# Autodesk Inventor assembly: Zusammengesetzt_2_Rechen_neu_3D
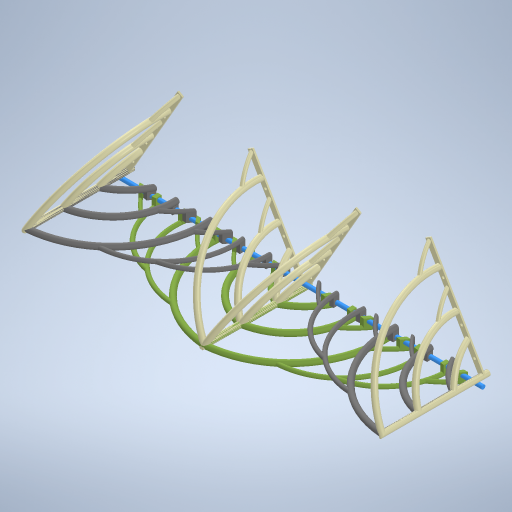
[picture p0: Inventor's stored thumbnail of the model, 512x512]
Saved by Autodesk Inventor 2024 (Build 280153000, 153)
## iProperties
Created: 2023-12-09
Part Number: Zusammengesetzt_2_Rechen_neu_3D
Document SubType Name: Assembly
Designer: mikao
Author: mikao
## Documents named in this file (5)
- \\192.168.122.200\studenten_bionik\Austausch\MikaOhler\Inventormodelle\Zusammengesetzt_2_Rechen_Stern_3D_Dickere_Wurzeln.iam
- \\192.168.122.200\studenten_bionik\Austausch\MikaOhler\Inventormodelle\schubsicherung_modul_links_Boden_glatt.ipt
- \\192.168.122.200\studenten_bionik\Austausch\MikaOhler\Inventormodelle\schubsicherung_modul_links_Boden_glatt_MIR.ipt
- \\192.168.122.200\studenten_bionik\Austausch\MikaOhler\Inventormodelle\schubsicherung_modul_links_Boden_glatt_Stütze.ipt
- \\192.168.122.200\studenten_bionik\Austausch\MikaOhler\Inventormodelle\Stange_4_Rechen.ipt
## Components (11 placed, 4 different names)
1. schubsicherung_modul_links_Boden_glatt:1 — Fluchtend:1, Starr:1
2. schubsicherung_modul_links_Boden_glatt:2 — Drehbar:1
3. schubsicherung_modul_links_Boden_glatt_MIR:1 — Passend:1, Drehbar:5
4. schubsicherung_modul_links_Boden_glatt_MIR:2 — Drehbar:3
5. schubsicherung_modul_links_Boden_glatt_Stütze:1 — Drehbar:1, Drehbar:2
6. schubsicherung_modul_links_Boden_glatt_Stütze:2 — Drehbar:4
7. Stange_4_Rechen:1 — Starr:1
8. schubsicherung_modul_links_Boden_glatt_Stütze:3 — Drehbar:2
9. schubsicherung_modul_links_Boden_glatt_Stütze:4 — Drehbar:3, Drehbar:4
10. schubsicherung_modul_links_Boden_glatt_Stütze:5 — Drehbar:5, Drehbar:6
11. schubsicherung_modul_links_Boden_glatt_Stütze:6 — Drehbar:6
## Relationships (9: RevoluteJoint 6, Flush 1, Mate 1, WeldJoint 1)
- Fluchtend:1 [Flush]: schubsicherung_modul_links_Boden_glatt:1
- Passend:1 [Mate]: schubsicherung_modul_links_Boden_glatt_MIR:1
- Starr:1 [WeldJoint] (54.55 mm): schubsicherung_modul_links_Boden_glatt:1 ↔ Stange_4_Rechen:1
- Drehbar:1 [RevoluteJoint]: schubsicherung_modul_links_Boden_glatt:2 ↔ schubsicherung_modul_links_Boden_glatt_Stütze:1
- Drehbar:2 [RevoluteJoint]: schubsicherung_modul_links_Boden_glatt_Stütze:1 ↔ schubsicherung_modul_links_Boden_glatt_Stütze:3
- Drehbar:3 [RevoluteJoint]: schubsicherung_modul_links_Boden_glatt_MIR:2 ↔ schubsicherung_modul_links_Boden_glatt_Stütze:4
- Drehbar:4 [RevoluteJoint]: schubsicherung_modul_links_Boden_glatt_Stütze:2 ↔ schubsicherung_modul_links_Boden_glatt_Stütze:4
- Drehbar:5 [RevoluteJoint]: schubsicherung_modul_links_Boden_glatt_MIR:1 ↔ schubsicherung_modul_links_Boden_glatt_Stütze:5
- Drehbar:6 [RevoluteJoint]: schubsicherung_modul_links_Boden_glatt_Stütze:5 ↔ schubsicherung_modul_links_Boden_glatt_Stütze:6
